# Autodesk Inventor assembly: ex8108
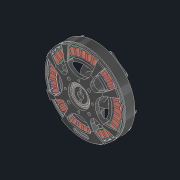
[picture p0: Inventor's stored thumbnail of the model, 180x180]
Saved by Autodesk Inventor 2021 (Build 250183000, 183)
## iProperties
Created: 2017-05-07
Part Number: ex8108
Document SubType Name: Assembly
Designer: Yuta Kage
Mass: 230 g
Surface Area: 488.185 cm^2
Volume: 53.0864 cm^3
Density: 4.33256 g/cm^3
Sending System: SolidWorks 2016
Last Author: Yureka
Last Saved: 2017-05-07
Author: Yuta Kage
## Documents named in this file (5)
- C:\Users\yuta0\Desktop\ZebraJointUnit\ex8108.iam
- C:\Users\yuta0\Documents\GitHub\zebra_hardware\hardware\mechanics\assy-zebra_ver1.0\020_U8_STATOR_HOUSING.ipt
- C:\Users\yuta0\Documents\GitHub\zebra_hardware\hardware\mechanics\assy-zebra_ver1.0\010_U8_ROTOR.ipt
- C:\Users\yuta0\Documents\GitHub\zebra_hardware\hardware\mechanics\assy-zebra_ver1.0\021_U8_STATOR_COILS.ipt
- C:\Users\yuta0\Documents\GitHub\zebra_hardware\hardware\mechanics\assy-zebra_ver1.0\5972K155_BALL BEARING.ipt
## Components (5 placed, 4 different names)
1. 020_U8_STATOR_HOUSING:1 — メイト:1, メイト:2, 角度:1, メイト:3, メイト:4
2. 010_U8_ROTOR:1 — メイト:1, メイト:2, 角度:1, メイト:5, メイト:6, メイト:7
3. 021_U8_STATOR_COILS:1 — メイト:3, メイト:4
4. 5972K155_BALL BEARING:1 — メイト:5, メイト:6
5. 5972K155_BALL BEARING:2 — メイト:7
## Relationships (8: Mate 7, Angle 1)
- メイト:1 [Mate] (-24.5 mm): 020_U8_STATOR_HOUSING:1 ↔ 010_U8_ROTOR:1
- メイト:2 [Mate]: 020_U8_STATOR_HOUSING:1 ↔ 010_U8_ROTOR:1
- 角度:1 [Angle] (0 deg): 020_U8_STATOR_HOUSING:1 ↔ 010_U8_ROTOR:1
- メイト:3 [Mate]: 020_U8_STATOR_HOUSING:1 ↔ 021_U8_STATOR_COILS:1
- メイト:4 [Mate]: 020_U8_STATOR_HOUSING:1 ↔ 021_U8_STATOR_COILS:1
- メイト:5 [Mate]: 010_U8_ROTOR:1 ↔ 5972K155_BALL BEARING:1
- メイト:6 [Mate]: 010_U8_ROTOR:1 ↔ 5972K155_BALL BEARING:1
- メイト:7 [Mate]: 010_U8_ROTOR:1 ↔ 5972K155_BALL BEARING:2
